# Autodesk Inventor assembly: DriveWheelCastingAssembly
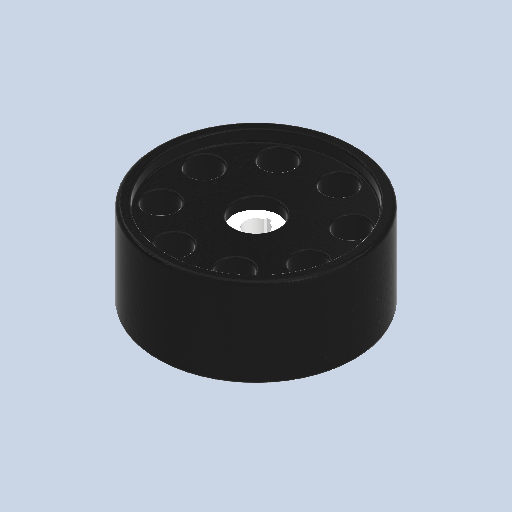
[picture p0: Inventor's stored thumbnail of the model, 512x512]
Saved by Autodesk Inventor 2022 (Build 260153000, 153)
## iProperties
Created: 2021-05-22
Part Number: DriveWheelCastingAssembly
Document SubType Name: Assembly
Designer: M3rob
Mass: 4034.57 g
Surface Area: 2993.02 cm^2
Volume: 3263.82 cm^3
Density: 1.23615 g/cm^3
Author: M3rob
## Documents named in this file (3)
- C:\Users\M3rob\Documents\GrabCAD\FireBird 250 Pound Gaming Machine\Drafts\FrameDrafts\Draft_04\Assemblies\DriveWheelCastingAssembly.iam
- C:\Users\M3rob\Documents\GrabCAD\FireBird 250 Pound Gaming Machine\Drafts\FrameDrafts\Draft_04\Drive\WheelHubMockup.ipt
- C:\Users\M3rob\Documents\GrabCAD\FireBird 250 Pound Gaming Machine\Drafts\FrameDrafts\Draft_04\Drive\CastWheel.ipt
## Components (2 placed, 2 different names)
1. WheelHubMockup:1 — Mate:1, Flush:1
2. CastWheel:1 — Mate:1, Flush:1
## Relationships (2: Mate 1, Flush 1)
- Mate:1: WheelHubMockup:1 ↔ CastWheel:1
- Flush:1 (-6.35 mm): WheelHubMockup:1 ↔ CastWheel:1
